# Autodesk Inventor assembly: phoenixcontact_0801733_din_rail
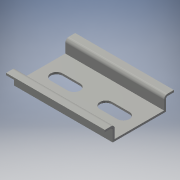
[picture p0: Inventor's stored thumbnail of the model, 180x180]
Saved by Autodesk Inventor 2018 (Build 220112000, 112)
## iProperties
Created: 2020-01-16
Part Number: phoenixcontact_0801733_din_rail
Description: Creo Elements/Direct Modeling STEP Export
Document SubType Name: Assembly
Designer: pollak
Sending System: Creo Elements/Direct Modeling 20.1A  29-Sep-2018 (C) Parametric Technology GmbH
Preprocessor: Creo Elements/Direct Modeling STEP processor for AP214 (Solid Model)
Title: C:/temp/JobSpoolerServerData/JobServer Files/59b414ee-d08b-4a31-b405-60fc9af73807/work/output/model.stp
## Documents named in this file (2)
- C:\Users\pollak\ownCloud\Inventor\ATA_2019\ATA_RFSoc_Enclosure\Parts\phoenixcontact_0801733_din_rail\phoenixcontact_0801733_din_rail.iam
- C:\Users\pollak\ownCloud\Inventor\ATA_2019\ATA_RFSoc_Enclosure\Parts\phoenixcontact_0801733_din_rail\NS_35_7.5_PERF_2000MM-select.ipt
## Components (2 placed, 2 different names)
1. 1 — Mate:1, Flush:1, Flush:2
2. NS_35_7.5_PERF_2000MM-select:2 — Mate:1, Flush:1, Flush:2
## Relationships (3: Flush 2, Mate 1)
- Mate:1: 1 ↔ NS_35_7.5_PERF_2000MM-select:2
- Flush:1: 1 ↔ NS_35_7.5_PERF_2000MM-select:2
- Flush:2: 1 ↔ NS_35_7.5_PERF_2000MM-select:2
